# Autodesk Inventor assembly: Dust Extractor_Assembly
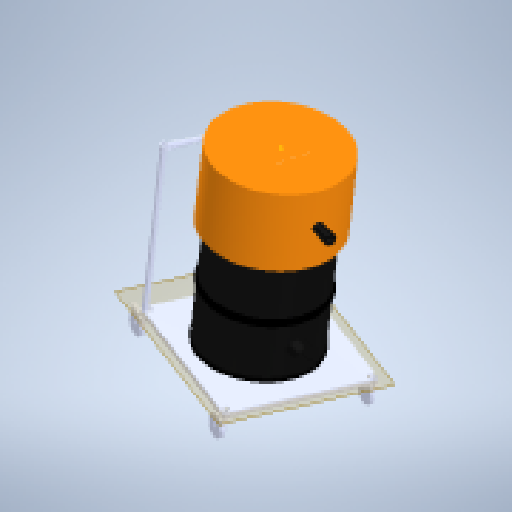
[picture p0: Inventor's stored thumbnail of the model, 512x512]
Saved by Autodesk Inventor 2025.2 (Build 292293000, 293)
## iProperties
Created: 2025-05-24
Part Number: Dust Extractor_Assembly
Document SubType Name: Assembly
Designer: Musa Gamal
Author: Musa Gamal
## Documents named in this file (3)
- D:\ASU\senior 1\semster 2\Advanced Manufacturing Technology & Prototyping\Project\Final Assembly\Project1\New folder (2)\Dust Extractor_Assembly.iam
- D:\ASU\senior 1\semster 2\Advanced Manufacturing Technology & Prototyping\Project\Final Assembly\Project1\New folder (2)\LUNYEE Dust Extractor.ipt
- D:\ASU\senior 1\semster 2\Advanced Manufacturing Technology & Prototyping\Project\Trolley\Trolley\Trolley.iam
## Components (2 placed, 2 different names)
1. LUNYEE Dust Extractor:1 — Mate:2, Mate:3
2. Trolley:1 [sub-assembly] — Mate:2, Mate:3
## Relationships (2: Mate 2)
- Mate:2: LUNYEE Dust Extractor:1 ↔ Trolley:1
- Mate:3: LUNYEE Dust Extractor:1 ↔ Trolley:1
